# Autodesk Inventor assembly: roller
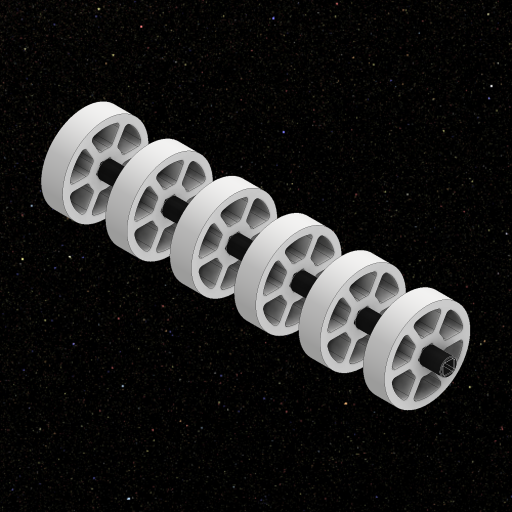
[picture p0: Inventor's stored thumbnail of the model, 512x512]
Saved by Autodesk Inventor 2024 (Build 280153000, 153)
## iProperties
Created: 2024-02-12
Part Number: roller
Document SubType Name: Assembly
Designer: Averey Ku
Author: Averey Ku
## Documents named in this file (5)
- D:\vex_robotics\hardware\cad\vroomba_v0.1\intake\roller.iam
- D:\vex_robotics\hardware\cad\VEX-CAD-Inventor-1.41\Motion\Wheels\Flex Wheels\2.000 Flex Wheel\2.000 30A .500.ipt
- D:\vex_robotics\hardware\cad\VEX-CAD-Inventor-1.41\Motion\Wheels\Flex Wheels\2.000 Flex Wheel.ipt
- D:\vex_robotics\hardware\cad\VEX-CAD-Inventor-1.41\Motion\Shaft HS\HS Spacer\HSpacer .5000.ipt
- D:\vex_robotics\hardware\cad\VEX-CAD-Inventor-1.41\Motion\Shaft HS\HS Spacer.ipt
## Components (18 placed, 2 different names)
1. 2.000 30A .500:1 — Insert:6, Insert:16
2. 2.000 30A .500:2 — Insert:7, Insert:8
3. 2.000 30A .500:3 — Insert:9, Insert:10
4. 2.000 30A .500:4 — Insert:11, Insert:12
5. 2.000 30A .500:5 — Insert:13, Insert:14
6. 2.000 30A .500:6 — Insert:15, Insert:17
7. HSpacer .5000:1 — Insert:1, Insert:6
8. HSpacer .5000:2 — Insert:1, Insert:7
9. HSpacer .5000:3 — Insert:14
10. HSpacer .5000:4 — Insert:15
11. HSpacer .5000:5 — Insert:12
12. HSpacer .5000:6 — Insert:13
13. HSpacer .5000:7 — Insert:10
14. HSpacer .5000:8 — Insert:11
15. HSpacer .5000:9 — Insert:8
16. HSpacer .5000:10 — Insert:9
17. HSpacer .5000:11 — Insert:17
18. HSpacer .5000:12 — Insert:16
## Relationships (17: Insert 17)
- Insert:1: HSpacer .5000:1 ↔ HSpacer .5000:2
- [Insert]: HSpacer .5000:3 ↔ HSpacer .5000:4
- [Insert]: HSpacer .5000:5 ↔ HSpacer .5000:6
- [Insert]: HSpacer .5000:7 ↔ HSpacer .5000:8
- [Insert]: HSpacer .5000:9 ↔ HSpacer .5000:10
- Insert:6: 2.000 30A .500:1 ↔ HSpacer .5000:1
- Insert:7: 2.000 30A .500:2 ↔ HSpacer .5000:2
- Insert:8: 2.000 30A .500:2 ↔ HSpacer .5000:9
- Insert:9: 2.000 30A .500:3 ↔ HSpacer .5000:10
- Insert:10: 2.000 30A .500:3 ↔ HSpacer .5000:7
- Insert:11: 2.000 30A .500:4 ↔ HSpacer .5000:8
- Insert:12: 2.000 30A .500:4 ↔ HSpacer .5000:5
- Insert:13: 2.000 30A .500:5 ↔ HSpacer .5000:6
- Insert:14: 2.000 30A .500:5 ↔ HSpacer .5000:3
- Insert:15: 2.000 30A .500:6 ↔ HSpacer .5000:4
- Insert:16: 2.000 30A .500:1 ↔ HSpacer .5000:12
- Insert:17: 2.000 30A .500:6 ↔ HSpacer .5000:11
## Named parameters: d1_d0 = 0 mm, d2_d0 = 0 mm, d3_d0 = 0 mm, d4_d0 = 0 mm
